# Autodesk Inventor assembly: conveyor
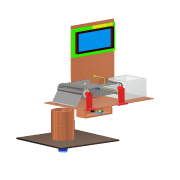
[picture p0: Inventor's stored thumbnail of the model, 180x180]
Saved by Autodesk Inventor 2021 (Build 250183000, 183)
## iProperties
Created: 2021-06-26
Part Number: conveyor
Document SubType Name: Assembly
Designer: Shaheen Khan
Author: Shaheen Khan
## Documents named in this file (22)
- C:\Users\Shaheen Khan\Desktop\inventor\conveyor.iam
- C:\Users\Shaheen Khan\Desktop\inventor\conveyor path.ipt
- C:\Users\Shaheen Khan\Desktop\inventor\12.ipt
- C:\Users\Shaheen Khan\Desktop\inventor\01.ipt
- C:\Users\Shaheen Khan\Desktop\inventor\as.ipt
- C:\Users\Shaheen Khan\Desktop\inventor\lllll.ipt
- C:\Users\Shaheen Khan\Desktop\inventor\gh.ipt
- C:\Users\Shaheen Khan\Desktop\inventor\baseee1.ipt
- C:\Users\Shaheen Khan\Downloads\lcd display (1).ipt
- C:\Users\Shaheen Khan\Documents\Inventor\Content Center Files\R2021\en-US\AS 1427(08)\AS 1427 - M5 x 16(6) I.ipt
- C:\Users\Shaheen Khan\Downloads\Box (1) (1).ipt
- C:\Users\Shaheen Khan\Desktop\inventor\sd.ipt
- C:\Users\Shaheen Khan\Desktop\inventor\servo.ipt
- C:\Users\Shaheen Khan\Downloads\ardUINO.ipt
- C:\Users\Shaheen Khan\Desktop\inventor\bracket1.ipt
- C:\Users\Shaheen Khan\Desktop\inventor\ab.ipt
- C:\Users\Shaheen Khan\Desktop\inventor\ghj.ipt
- C:\Users\Shaheen Khan\Desktop\inventor\aa.ipt
- C:\Users\Shaheen Khan\Desktop\inventor\abb.ipt
- C:\Users\Shaheen Khan\Desktop\inventor\buzz.ipt
- C:\Users\Shaheen Khan\Documents\Inventor\Content Center Files\R2021\en-US\SFS 2976\SFS 2976 - M5 x 16.ipt
- C:\Users\Shaheen Khan\Desktop\inventor\wer.ipt
## Components (92 placed, 21 different names)
1. conveyor path:1 — Flush:1, Flush:2, Flush:3, Mate:3, Mate:4, Mate:38
2. as:1 — Mate:5, Mate:8
3. as:2 — Mate:6, Mate:9
4. lllll:1 — Mate:8, Mate:20
5. lllll:2 — Mate:7, Mate:20
6. gh:1 — Mate:9, Mate:19, Mate:21, Mate:22, Mate:23
7. gh:2 — Mate:10, Mate:19
8. baseee1:1 — Mate:11, Mate:12, Mate:13, Mate:21, Mate:22, Mate:23, Mate:24, Mate:25, Mate:34
9. lcd display (1):1 — Mate:11, Mate:12, Mate:13, Mate:14, Mate:15, Mate:16, Mate:17
10. AS 1427 Z - Metric M5 x 16:4 — Mate:14
11. AS 1427 Z - Metric M5 x 16:5 — Mate:16
12. AS 1427 Z - Metric M5 x 16:6 — Mate:17
13. AS 1427 Z - Metric M5 x 16:7 — Mate:15
14. Box (1) (1):1 — Mate:24, Mate:25
15. sd:1 — Mate:28
16. ardUINO:1 — Mate:31
17. bracket1:1 — Mate:31, Mate:33, Mate:34, Mate:41
18. ab:1 — Mate:32
19. ghj:1 — Mate:33
20. servo:1 — Mate:35, Mate:36, Mate:39, Mate:42, Mate:43, Mate:44, Mate:45, Angle:2, Mate:46
21. aa:1 — Mate:35, Mate:36, Mate:40, Angle:2
22. abb:1 — Mate:38
23. buzz:1 — Mate:41
24. SFS 2976 M5 x 16:3 — Mate:42
25. SFS 2976 M5 x 16:4 — Mate:43
26. SFS 2976 M5 x 16:5 — Mate:44
27. SFS 2976 M5 x 16:6 — Mate:45
28. wer:1 — Mate:46
29. 12:1 — Mate:1, Mate:2, Angle:1, Mate:5, Mate:10
30. 12:2 — Mate:6, Mate:7
31. 01:1 — Mate:3
32. 01:2
33. 01:3
34. 01:4
35. 01:5
36. 01:6
37. 01:7 — Mate:28
38. 01:8
39. 01:9
40. 01:10
41. 01:11
42. 01:12
43. 01:13
44. 01:14
45. 01:15
46. 01:16
47. 01:17
48. 01:18
49. 01:19
50. 01:20
51. 01:21
52. 01:22
53. 01:23
54. 01:24
55. 01:25
56. 01:26
57. 01:27
58. 01:28
59. 01:29
60. 01:30
61. 01:31
62. 01:32
63. 01:33
64. 01:34
65. 01:35
66. 01:36
67. 01:37
68. 01:38
69. 01:39
70. 01:40
71. 01:41
72. 01:42
73. 01:43
74. 01:44
75. 01:45
76. 01:46
77. 01:47
78. 01:48
79. 01:49
80. 01:50
81. 01:51
82. 01:52
83. 01:53
84. 01:54
85. 01:55 — Mate:32
86. 01:56
87. 01:57
88. 01:58
89. 01:59
90. 01:60
91. 01:61
92. 01:62
## Component patterns: (2 elements, first: 12:1), (62 elements, first: 01:1)
## Relationships (45: Mate 40, Flush 3, Angle 2)
- Flush:1: conveyor path:1
- Flush:2: conveyor path:1
- Flush:3: conveyor path:1
- Mate:1: 12:1
- Mate:2: 12:1
- Mate:3: conveyor path:1 ↔ 01:1
- Mate:4 (300.1 mm): conveyor path:1
- Angle:1 (0 deg): 12:1
- Mate:5: as:1 ↔ 12:1
- Mate:6: as:2 ↔ 12:2
- Mate:7: lllll:2 ↔ 12:2
- Mate:8: as:1 ↔ lllll:1
- Mate:9: as:2 ↔ gh:1
- Mate:10: gh:2 ↔ 12:1
- Mate:11: baseee1:1 ↔ lcd display (1):1
- Mate:12: baseee1:1 ↔ lcd display (1):1
- Mate:13: baseee1:1 ↔ lcd display (1):1
- Mate:14: lcd display (1):1 ↔ AS 1427 Z - Metric M5 x 16:4
- Mate:15: lcd display (1):1 ↔ AS 1427 Z - Metric M5 x 16:7
- Mate:16: lcd display (1):1 ↔ AS 1427 Z - Metric M5 x 16:5
- Mate:17: lcd display (1):1 ↔ AS 1427 Z - Metric M5 x 16:6
- Mate:19: gh:1 ↔ gh:2
- Mate:20: lllll:1 ↔ lllll:2
- Mate:21: gh:1 ↔ baseee1:1
- Mate:22: gh:1 ↔ baseee1:1
- Mate:23 (-120 mm): gh:1 ↔ baseee1:1
- Mate:24: baseee1:1 ↔ Box (1) (1):1
- Mate:25 (-10 mm): baseee1:1 ↔ Box (1) (1):1
- Mate:28: sd:1 ↔ 01:7
- Mate:31: ardUINO:1 ↔ bracket1:1
- Mate:32: ab:1 ↔ 01:55
- Mate:33: bracket1:1 ↔ ghj:1
- Mate:34: baseee1:1 ↔ bracket1:1
- Mate:35: servo:1 ↔ aa:1
- Mate:36: servo:1 ↔ aa:1
- Mate:38 (200 mm): conveyor path:1 ↔ abb:1
- Mate:39: servo:1
- Mate:40 (100 mm): aa:1
- Mate:41: bracket1:1 ↔ buzz:1
- Mate:42: servo:1 ↔ SFS 2976 M5 x 16:3
- Mate:43: servo:1 ↔ SFS 2976 M5 x 16:4
- Mate:44: servo:1 ↔ SFS 2976 M5 x 16:5
- Mate:45: servo:1 ↔ SFS 2976 M5 x 16:6
- Angle:2 (90 deg): servo:1 ↔ aa:1
- Mate:46: servo:1 ↔ wer:1
